# Autodesk Inventor assembly: PCBAssemblyFEA
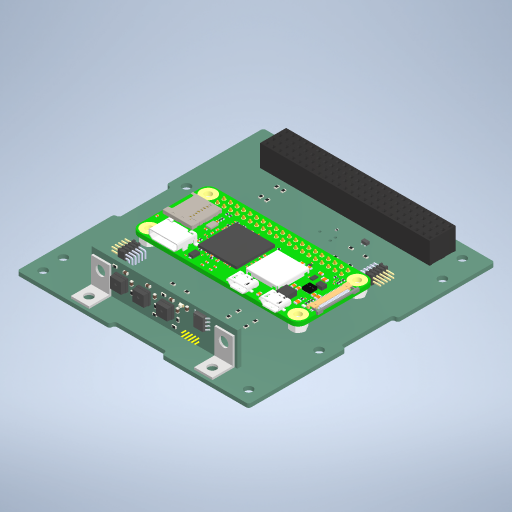
[picture p0: Inventor's stored thumbnail of the model, 512x512]
Saved by Autodesk Inventor 2023.5 (Build 275446020, 446B)
## iProperties
Created: 2026-07-20
Part Number: PCBAssemblyFEA
Document SubType Name: Assembly
Designer: User
Author: User
## Documents named in this file (6)
- C:\Users\User\Projects\missionpegasusPCB\CAD\PCBAssemblyFEA.iam
- C:\Users\User\Projects\missionpegasusPCB\CAD\615Bracket.ipt
- C:\Users\User\Downloads\User Library-40-pin GPIO Header for Raspberry Pi (color-coded)\User Library-40-pin GPIO Header for Raspberry Pi (color-coded).ipt
- C:\Users\User\Downloads\LIB_R25-3000302\R25-3000302\3D\R25-3000302\R25-3000302.ipt
- C:\Users\User\Projects\missionpegasusPCB\mezzanine-board\sensorboard5\sensorboard5.ipt
- C:\Users\User\Projects\missionpegasusPCB\main-board\mainboard6\mainboard6.ipt
## Components (9 placed, 5 different names)
1. User Library-40-pin GPIO Header for Raspberry Pi (color-coded):1 — Mate:23
2. R25-3000302:1 — Mate:22
3. R25-3000302:2 — Mate:19
4. R25-3000302:3 — Mate:20
5. R25-3000302:4 — Mate:21
6. 615Bracket:18 — Mate:16, Mate:17
7. 615Bracket:19 — Mate:18
8. sensorboard5:5 — Mate:16
9. mainboard6:1 — Mate:17, Mate:18, Mate:19, Mate:20, Mate:21, Mate:22, Mate:23
## Relationships (8: Mate 8)
- Mate:16: 615Bracket:18 ↔ sensorboard5:5
- Mate:17: 615Bracket:18 ↔ mainboard6:1
- Mate:18: 615Bracket:19 ↔ mainboard6:1
- Mate:19: R25-3000302:2 ↔ mainboard6:1
- Mate:20: R25-3000302:3 ↔ mainboard6:1
- Mate:21: R25-3000302:4 ↔ mainboard6:1
- Mate:22: R25-3000302:1 ↔ mainboard6:1
- Mate:23: User Library-40-pin GPIO Header for Raspberry Pi (color-coded):1 ↔ mainboard6:1
